# Autodesk Inventor assembly: COTS_Pasternack_RG58CU_Coax_Cable
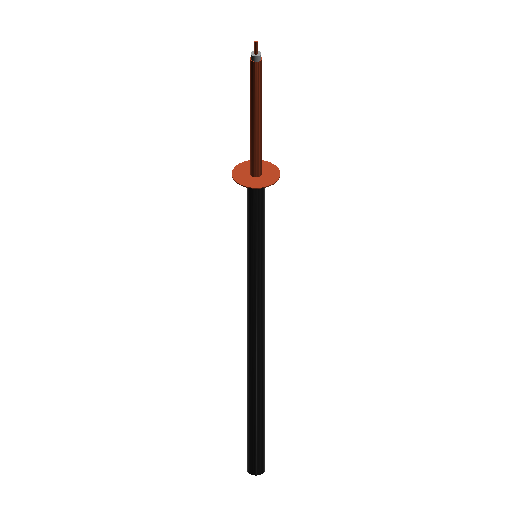
[picture p0: Inventor's stored thumbnail of the model, 512x512]
Saved by Autodesk Inventor 2026 (Build 300175000, 175)
## iProperties
Part Number: COTS_Pasternack_RG58CU_Coax_Cable
Document SubType Name: Assembly
Designer: User
Author: User
## Documents named in this file (5)
- D:\_ANDRZEJ_LACZEWSKI\_OTHER\RF - Mostly 3D Printed Discone Antenna\MCAD\15_DISCONE_V4\__COTS_PARTS\COTS_Pasternack_RG58CU_Coax_Cable\COTS_Pasternack_RG58CU_Coax_Cable.iam
- D:\_ANDRZEJ_LACZEWSKI\_OTHER\RF - Mostly 3D Printed Discone Antenna\MCAD\15_DISCONE_V4\__COTS_PARTS\COTS_Pasternack_RG58CU_Coax_Cable\Outer_Jacket.ipt
- D:\_ANDRZEJ_LACZEWSKI\_OTHER\RF - Mostly 3D Printed Discone Antenna\MCAD\15_DISCONE_V4\__COTS_PARTS\COTS_Pasternack_RG58CU_Coax_Cable\Shield.ipt
- D:\_ANDRZEJ_LACZEWSKI\_OTHER\RF - Mostly 3D Printed Discone Antenna\MCAD\15_DISCONE_V4\__COTS_PARTS\COTS_Pasternack_RG58CU_Coax_Cable\Dielectric.ipt
- D:\_ANDRZEJ_LACZEWSKI\_OTHER\RF - Mostly 3D Printed Discone Antenna\MCAD\15_DISCONE_V4\__COTS_PARTS\COTS_Pasternack_RG58CU_Coax_Cable\Inner_Conductor.ipt
## Components (4 placed, 4 different names)
1. Outer_Jacket:1 — Mate:1, Flush:1
2. Shield:1 — Mate:1, Flush:1, Mate:2, Flush:2
3. Dielectric:1 — Mate:2, Flush:2, Mate:3, Flush:3
4. Inner_Conductor:1 — Mate:3, Flush:3
## Relationships (6: Mate 3, Flush 3)
- Mate:1: Outer_Jacket:1 ↔ Shield:1
- Flush:1: Outer_Jacket:1 ↔ Shield:1
- Mate:2: Shield:1 ↔ Dielectric:1
- Flush:2: Shield:1 ↔ Dielectric:1
- Mate:3: Dielectric:1 ↔ Inner_Conductor:1
- Flush:3: Dielectric:1 ↔ Inner_Conductor:1
